# Autodesk Inventor assembly: 右前脚ユニット4
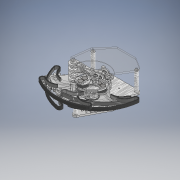
[picture p0: Inventor's stored thumbnail of the model, 180x180]
Saved by Autodesk Inventor 2020 (Build 240168000, 168)
## iProperties
Created: 2019-08-30
Part Number: 右前脚ユニット4
Document SubType Name: Assembly
Designer: 雪村
Mass: 235.188 g
Surface Area: 1182 cm^2
Volume: 114.039 cm^3
Density: 2.06235 g/cm^3
Author: 雪村
## Documents named in this file (13)
- C:\Users\white\Documents\SRDC\SRDC\Inventor_2017\2018年機体\2020年4年機体\右前脚ユニット4.iam
- C:\Users\white\Documents\SRDC\SRDC\Inventor_2017\2018年機体\2020年4年機体\脚外フレーム3_MIR.ipt
- C:\Users\white\Documents\SRDC\SRDC\Inventor_2017\2018年機体\2020年4年機体\脚内フレーム4_MIR.ipt
- C:\Users\white\Documents\SRDC\SRDC\Inventor_2017\2018年機体\2020年4年機体\脚クランク1.iam
- C:\Users\white\Documents\SRDC\SRDC\Inventor_2017\2018年機体\2020年4年機体\脚最終段カム1.ipt
- C:\Users\white\Documents\SRDC\SRDC\Inventor_2017\2018年機体\パーツ\オイレスフランジ付き12142006.ipt
- C:\Users\white\Documents\SRDC\SRDC\Inventor_2017\2018年機体\パーツ\スペーサーm3,35.ipt
- C:\Users\white\Documents\SRDC\SRDC\Inventor_2017\2018年機体\2020年4年機体\ヘッケン＋揺動節1.iam
- C:\Users\white\Documents\SRDC\SRDC\Inventor_2017\2018年機体\2020年4年機体\歯車m2.z21.2.ipt
- C:\Users\white\Documents\SRDC\SRDC\Inventor_2017\2018年機体\2020年4年機体\脚最終段抑え1.ipt
- C:\Users\white\Documents\SRDC\SRDC\Inventor_2017\2018年機体\パーツ\スペーサーm3,11.ipt
- C:\Users\white\Documents\SRDC\SRDC\Inventor_2017\2018年機体\2020年4年機体\脚最終段カム2.ipt
- C:\Users\white\Documents\SRDC\SRDC\Inventor_2017\2018年機体\2020年4年機体\前脚ギアトレイン3_MIR.iam
## Components (20 placed, 12 different names)
1. 脚外フレーム3_MIR:1
2. 脚内フレーム4_MIR:1 — 挿入:24
3. 脚クランク1:1 [sub-assembly]
4. 脚最終段カム1:1
5. オイレスフランジ付き12142006:1
6. スペーサーm3,35:1
7. スペーサーm3,35:2
8. スペーサーm3,35:3
9. ヘッケン＋揺動節1:1 [sub-assembly]
10. ヘッケン＋揺動節1:2 [sub-assembly]
11. ヘッケン＋揺動節1:3 [sub-assembly]
12. ヘッケン＋揺動節1:4 [sub-assembly]
13. 歯車m2.z21.2:1
14. 脚最終段抑え1:1
15. スペーサーm3,11:1
16. スペーサーm3,11:2
17. スペーサーm3,11:3
18. 脚最終段カム2:1
19. オイレスフランジ付き12142006:2
20. 前脚ギアトレイン3_MIR:1 [sub-assembly] — 挿入:24
## Relationships (28: Insert 24, Mate 4)
- [Insert]: 脚クランク1:1 ↔ 脚最終段カム1:1
- [Insert]: 脚クランク1:1 ↔ 脚最終段カム1:1
- [Insert]: 脚最終段カム1:1 ↔ オイレスフランジ付き12142006:1
- [Insert] (0.5 mm): 脚クランク1:1 ↔ ヘッケン＋揺動節1:4
- [Insert] (0.5 mm): 脚クランク1:1 ↔ ヘッケン＋揺動節1:3
- [Insert] (0.5 mm): 脚クランク1:1 ↔ ヘッケン＋揺動節1:2
- [Insert] (0.5 mm): 脚クランク1:1 ↔ ヘッケン＋揺動節1:1
- [Mate]: スペーサーm3,35:3 ↔ ヘッケン＋揺動節1:3
- [Mate]: スペーサーm3,35:3 ↔ ヘッケン＋揺動節1:4
- [Mate]: スペーサーm3,35:3 ↔ ヘッケン＋揺動節1:2
- [Mate]: スペーサーm3,35:3 ↔ ヘッケン＋揺動節1:1
- [Insert]: 脚最終段カム1:1 ↔ 歯車m2.z21.2:1
- [Insert]: 脚最終段カム1:1 ↔ 歯車m2.z21.2:1
- [Insert]: 脚内フレーム4_MIR:1 ↔ スペーサーm3,35:3
- [Insert]: 脚内フレーム4_MIR:1 ↔ オイレスフランジ付き12142006:1
- [Insert]: 脚内フレーム4_MIR:1 ↔ スペーサーm3,35:1
- [Insert]: 脚内フレーム4_MIR:1 ↔ スペーサーm3,35:2
- [Insert]: 脚外フレーム3_MIR:1 ↔ スペーサーm3,35:3
- [Insert]: 脚外フレーム3_MIR:1 ↔ スペーサーm3,35:1
- [Insert]: 脚最終段抑え1:1 ↔ スペーサーm3,11:2
- [Insert]: 脚最終段抑え1:1 ↔ スペーサーm3,11:1
- [Insert]: 脚最終段抑え1:1 ↔ スペーサーm3,11:3
- [Insert]: 脚内フレーム4_MIR:1 ↔ スペーサーm3,11:3
- [Insert]: 脚内フレーム4_MIR:1 ↔ スペーサーm3,11:2
- [Insert]: 歯車m2.z21.2:1 ↔ 脚最終段カム2:1
- [Insert]: 歯車m2.z21.2:1 ↔ 脚最終段カム2:1
- [Insert]: 脚最終段カム2:1 ↔ オイレスフランジ付き12142006:2
- 挿入:24 [Insert]: 脚内フレーム4_MIR:1 ↔ 前脚ギアトレイン3_MIR:1
## Named parameters: d8_d21 = 0 mm, d11_d12 = 0 mm, d10_d13 = 0 mm, d3_d10 = 0.5 mm, d4_d11 = 0 mm, d5_d12 = 0 mm, d16_d20 = 0 mm
